# Autodesk Inventor assembly: Arm
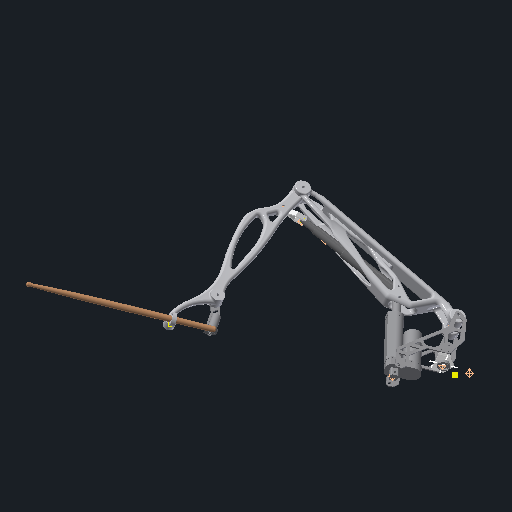
[picture p0: Inventor's stored thumbnail of the model, 512x512]
Saved by Autodesk Inventor 2025.2 (Build 292293000, 293)
## iProperties
Created: 2020-03-24
Part Number: Arm
Document SubType Name: Assembly
Designer: valer
Mass: 4853.13 g
Surface Area: 3141.52 cm^2
Volume: 1403.99 cm^3
Density: 3.45667 g/cm^3
Author: valer
## Documents named in this file (11)
- C:\Users\valer\Desktop\str1ker\cad\Arm.iam
- C:\Users\valer\Desktop\str1ker\cad\UpperArm.iam
- C:\Users\valer\Desktop\str1ker\cad\Forearm.iam
- C:\Users\valer\Desktop\str1ker\cad\Drumstick.iam
- C:\Users\valer\Desktop\str1ker\cad\ArmSolenoid.iam
- C:\Users\valer\Desktop\str1ker\cad\external\UpperArmActuator\UpperArmActuatorBase.iam
- C:\Users\valer\Desktop\str1ker\cad\external\UpperArmActuator\UpperArmActuatorShaft.iam
- C:\Users\valer\Desktop\str1ker\cad\external\ForearmActuator\ForearmActuatorBody.iam
- C:\Users\valer\Desktop\str1ker\cad\ForearmActuatorConnector.iam
- C:\Users\valer\Desktop\str1ker\cad\external\ForearmActuator\ForearmActuatorShaft.iam
- C:\Users\valer\Desktop\str1ker\cad\ShoulderRedesign.iam
## Components (10 placed, 10 different names)
1. UpperArm:1 [sub-assembly] — Mate:6, Mate:7, Mate:29, Flush:3, Mate:30, Mate:35, Mate:36
2. Forearm:1 [sub-assembly] — Mate:6, Mate:7, Mate:8, Mate:9, Mate:10, Mate:11, Mate:31
3. Drumstick:1 [sub-assembly] — Mate:8, Mate:9
4. ArmSolenoid:1 [sub-assembly] — Mate:10, Mate:11
5. UpperArmActuatorBase:1 [sub-assembly] — Mate:28, Mate:37, Mate:38
6. UpperArmActuatorShaft:1 [sub-assembly] — Mate:28, Mate:29
7. ForearmActuatorBody:1 [sub-assembly] — Flush:3, Mate:30, Mate:32, Mate:33
8. ForearmActuatorConnector:1 [sub-assembly] — Mate:31, Mate:32, Mate:34
9. ForearmActuatorShaft:1 [sub-assembly] — Mate:33, Mate:34
10. Shoulder:1 [sub-assembly] — Mate:35, Mate:36, Mate:37, Mate:38
## Relationships (18: Mate 17, Flush 1)
- Mate:6: UpperArm:1 ↔ Forearm:1
- Mate:7: UpperArm:1 ↔ Forearm:1
- Mate:8: Forearm:1 ↔ Drumstick:1
- Mate:9: Forearm:1 ↔ Drumstick:1
- Mate:10: Forearm:1 ↔ ArmSolenoid:1
- Mate:11: Forearm:1 ↔ ArmSolenoid:1
- Mate:28: UpperArmActuatorBase:1 ↔ UpperArmActuatorShaft:1
- Mate:29: UpperArm:1 ↔ UpperArmActuatorShaft:1
- Flush:3: UpperArm:1 ↔ ForearmActuatorBody:1
- Mate:30: UpperArm:1 ↔ ForearmActuatorBody:1
- Mate:31: Forearm:1 ↔ ForearmActuatorConnector:1
- Mate:32: ForearmActuatorBody:1 ↔ ForearmActuatorConnector:1
- Mate:33: ForearmActuatorBody:1 ↔ ForearmActuatorShaft:1
- Mate:34: ForearmActuatorConnector:1 ↔ ForearmActuatorShaft:1
- Mate:35: UpperArm:1 ↔ Shoulder:1
- Mate:36: UpperArm:1 ↔ Shoulder:1
- Mate:37: UpperArmActuatorBase:1 ↔ Shoulder:1
- Mate:38 (20 mm): UpperArmActuatorBase:1 ↔ Shoulder:1
